# Autodesk Inventor assembly: Marco_apm_002-3
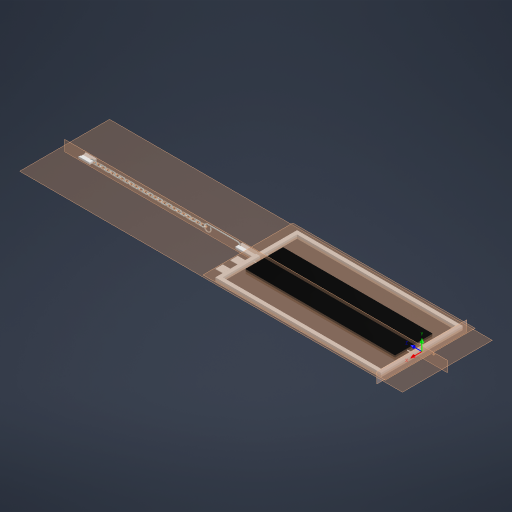
[picture p0: Inventor's stored thumbnail of the model, 512x512]
Saved by Autodesk Inventor 2024 (Build 280153000, 153)
## iProperties
Created: 2023-05-17
Part Number: Marco_apm_002-3
Document SubType Name: Assembly
Designer: javie
Author: javie
## Documents named in this file (7)
- C:\Users\javie\Downloads\Piezas CMR\Marco_APM_002\Marco_apm_002-3.iam
- C:\Users\javie\Downloads\Piezas CMR\Marco_Conveyor_Aereo.iam
- C:\Users\javie\Downloads\Piezas CMR\Marcos_solids\Pieza1.ipt
- C:\Users\javie\Downloads\Piezas CMR\Marcos_solids\Pieza2.ipt
- C:\Users\javie\Downloads\Piezas CMR\Marco_APM_002\Piezas\APM_002-3.ipt
- C:\Users\javie\Downloads\Piezas CMR\Marcos_solids\Topes_apm_002-2.ipt
- C:\Users\javie\Downloads\Piezas CMR\S_RobotStudio_Model\Pieza3.ipt
## Components (6 placed, 6 different names)
1. Marco_Conveyor_Aereo:1 [sub-assembly] — Nivelación:1, Nivelación:2, Nivelación:3
2. Pieza1:1 — Nivelación:1, Insertar:1
3. Pieza2:1
4. APM_002-3:1 — Insertar:1, Insertar:2, Insertar:3
5. Topes_apm_002-2:1 — Insertar:2, Insertar:3
6. Pieza3:1 — Nivelación:2, Nivelación:3
## Relationships (6: Flush 3, Insert 3)
- Nivelación:1 [Flush]: Marco_Conveyor_Aereo:1 ↔ Pieza1:1
- Insertar:1: Pieza1:1 ↔ APM_002-3:1
- Insertar:2: APM_002-3:1 ↔ Topes_apm_002-2:1
- Insertar:3: APM_002-3:1 ↔ Topes_apm_002-2:1
- Nivelación:2 [Flush]: Marco_Conveyor_Aereo:1 ↔ Pieza3:1
- Nivelación:3 [Flush]: Marco_Conveyor_Aereo:1 ↔ Pieza3:1
